# Autodesk Inventor assembly: Chain-ver1-1111-2018
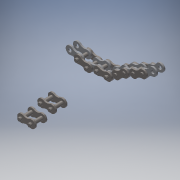
[picture p0: Inventor's stored thumbnail of the model, 180x180]
Saved by Autodesk Inventor 2017 (Build 210142000, 142)
## iProperties
Created: 2018-01-27
Part Number: Chain-ver1-1111-2018
Document SubType Name: Assembly
Designer: 764368
Author: 764368
## Documents named in this file (4)
- E:\GrabCAD\Power Hawks CAD\VEXpro Resources\Versa Motion\Chain\Chain-ver1-1111-2018.iam
- E:\GrabCAD\Power Hawks CAD\VEXpro Resources\Versa Motion\Chain\MasterChain-1111-2018.ipt
- E:\GrabCAD\Power Hawks CAD\VEXpro Resources\Versa Motion\Chain\ChainInterLink-ver1-1111-2018.iam
- E:\GrabCAD\Power Hawks CAD\VEXpro Resources\Versa Motion\Chain\LockCHain-ver1-1111-2018.ipt
## Components (18 placed, 3 different names)
1. LockCHain-ver1-1111-2018:1 — Rotational:1, Rotational:3
2. ChainInterLink-ver1-1111-2018:1 [sub-assembly] — Rotational:3, Rotational:4
3. ChainInterLink-ver1-1111-2018:2 [sub-assembly] — Rotational:1, Rotational:2
4. ChainInterLink-ver1-1111-2018:3 [sub-assembly] — Rotational:5
5. ChainInterLink-ver1-1111-2018:4 [sub-assembly] — Rotational:6, Rotational:7
6. ChainInterLink-ver1-1111-2018:5 [sub-assembly] — Rotational:8
7. MasterChain-1111-2018:1 — Rotational:7, Rotational:8
8. MasterChain-1111-2018:2
9. MasterChain-1111-2018:3
10. MasterChain-1111-2018:4
11. MasterChain-1111-2018:5
12. MasterChain-1111-2018:6
13. MasterChain-1111-2018:7
14. MasterChain-1111-2018:8
15. MasterChain-1111-2018:9
16. MasterChain-1111-2018:10 — Rotational:4, Rotational:5
17. MasterChain-1111-2018:11 — Rotational:2, Rotational:6
18. MasterChain-1111-2018:12
## Relationships (8: RevoluteJoint 8)
- Rotational:1 [RevoluteJoint]: LockCHain-ver1-1111-2018:1 ↔ ChainInterLink-ver1-1111-2018:2
- Rotational:2 [RevoluteJoint]: ChainInterLink-ver1-1111-2018:2 ↔ MasterChain-1111-2018:11
- Rotational:3 [RevoluteJoint]: LockCHain-ver1-1111-2018:1 ↔ ChainInterLink-ver1-1111-2018:1
- Rotational:4 [RevoluteJoint]: ChainInterLink-ver1-1111-2018:1 ↔ MasterChain-1111-2018:10
- Rotational:5 [RevoluteJoint]: ChainInterLink-ver1-1111-2018:3 ↔ MasterChain-1111-2018:10
- Rotational:6 [RevoluteJoint]: ChainInterLink-ver1-1111-2018:4 ↔ MasterChain-1111-2018:11
- Rotational:7 [RevoluteJoint]: ChainInterLink-ver1-1111-2018:4 ↔ MasterChain-1111-2018:1
- Rotational:8 [RevoluteJoint]: ChainInterLink-ver1-1111-2018:5 ↔ MasterChain-1111-2018:1
